# Autodesk Inventor assembly: insertAssembly-2
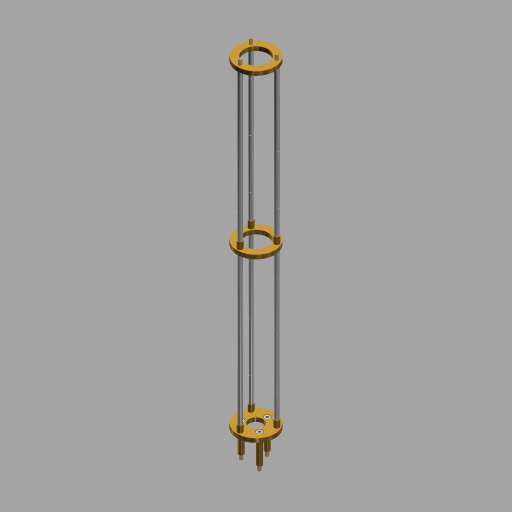
[picture p0: Inventor's stored thumbnail of the model, 512x512]
Saved by Autodesk Inventor 2024 (Build 280153020, 153B)
## iProperties
Created: 2023-09-24
Part Number: insertAssembly-2
Document SubType Name: Assembly
Designer: schanen
Author: schanen
## Documents named in this file (6)
- C:\Users\schanen\Documents\Inventor\he4inserts\insertAssembly-2.iam
- C:\Users\schanen\Documents\Inventor\he4inserts\CompositeSupport.iam
- C:\Users\schanen\Documents\Inventor\he4inserts\Insert_flange.ipt
- C:\Users\schanen\Documents\Inventor\he4inserts\Insert_flange_Top.ipt
- C:\Users\schanen\Documents\Inventor\he4inserts\Screw_StainlessSteal_M3_SocketCap_6mm.ipt
- C:\Users\schanen\Documents\Inventor\he4inserts\Fitting-3.ipt
## Components (18 placed, 5 different names)
1. Insert_flange:1 — Mate:9, Mate:10, Mate:11, Mate:17
2. Insert_flange_Top:1 — Mate:5, Mate:6, Mate:7, Mate:8, Mate:12, Mate:13, Mate:14, Mate:15
3. Insert_flange:2 — Mate:18, Mate:19, Mate:20
4. Fitting-3:1 [sub-assembly] — Mate:12, Mate:13
5. Screw_StainlessSteal_M3_SocketCap_6mm:1 — Mate:14, Mate:15
6. Fitting-3:2 [sub-assembly]
7. Screw_StainlessSteal_M3_SocketCap_6mm:2
8. Fitting-3:3 [sub-assembly]
9. Screw_StainlessSteal_M3_SocketCap_6mm:3
10. Screw_StainlessSteal_M3_SocketCap_6mm:4 — Mate:7, Mate:8
11. CompositeSupport:1 [sub-assembly] — Mate:5, Mate:6, Mate:16
12. Screw_StainlessSteal_M3_SocketCap_6mm:5
13. CompositeSupport:2 [sub-assembly] — Mate:10
14. Screw_StainlessSteal_M3_SocketCap_6mm:6
15. CompositeSupport:3 [sub-assembly] — Mate:9, Mate:11
16. CompositeSupport:4 [sub-assembly] — Mate:16, Mate:17, Mate:19, Mate:20
17. CompositeSupport:5 [sub-assembly] — Mate:18
18. CompositeSupport:6 [sub-assembly]
## Component patterns: (3 elements, first: Fitting-3:1 + Screw_StainlessSteal_M3_SocketCap_6mm:1), (3 elements, first: Screw_StainlessSteal_M3_SocketCap_6mm:4 + CompositeSupport:1), (3 elements, first: CompositeSupport:4)
## Relationships (16: Mate 16)
- Mate:5: Insert_flange_Top:1 ↔ CompositeSupport:1
- Mate:6: Insert_flange_Top:1 ↔ CompositeSupport:1
- Mate:7: Insert_flange_Top:1 ↔ Screw_StainlessSteal_M3_SocketCap_6mm:4
- Mate:8: Insert_flange_Top:1 ↔ Screw_StainlessSteal_M3_SocketCap_6mm:4
- Mate:9: Insert_flange:1 ↔ CompositeSupport:3
- Mate:10: Insert_flange:1 ↔ CompositeSupport:2
- Mate:11: Insert_flange:1 ↔ CompositeSupport:3
- Mate:12: Insert_flange_Top:1 ↔ Fitting-3:1
- Mate:13: Insert_flange_Top:1 ↔ Fitting-3:1
- Mate:14: Insert_flange_Top:1 ↔ Screw_StainlessSteal_M3_SocketCap_6mm:1
- Mate:15: Insert_flange_Top:1 ↔ Screw_StainlessSteal_M3_SocketCap_6mm:1
- Mate:16: CompositeSupport:1 ↔ CompositeSupport:4
- Mate:17: Insert_flange:1 ↔ CompositeSupport:4
- Mate:18: Insert_flange:2 ↔ CompositeSupport:5
- Mate:19: Insert_flange:2 ↔ CompositeSupport:4
- Mate:20: Insert_flange:2 ↔ CompositeSupport:4
